# Autodesk Inventor assembly: 部件1
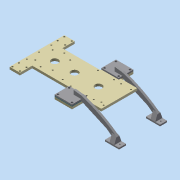
[picture p0: Inventor's stored thumbnail of the model, 180x180]
Saved by Autodesk Inventor 2019 (Build 230136000, 136)
## iProperties
Created: 2020-12-08
Part Number: 部件1
Document SubType Name: Assembly
Designer: Wang Hua
Author: Wang Hua
## Documents named in this file (5)
- C:\Users\Wang Hua\Documents\Inventor\机器人实践\装配文件\部件1.iam
- C:\Users\Wang Hua\Documents\Inventor\机器人实践\装配文件\左侧外部机械44mm.ipt
- C:\Users\Wang Hua\Documents\Inventor\机器人实践\装配文件\约135底盘4.0.ipt
- C:\Users\Wang Hua\Documents\Inventor\机器人实践\装配文件\自制垫片.ipt
- C:\Users\Wang Hua\Documents\Inventor\机器人实践\装配文件\右侧外部机械44mm.ipt
## Components (4 placed, 4 different names)
1. 左侧外部机械44mm:1 — 配合:1, 配合:2, 配合:3
2. 约135底盘4.0:1 — 配合:1, 配合:2, 配合:3, 配合:4, 配合:5, 配合:6
3. 自制垫片:1 — 配合:4, 配合:5, 配合:6, 配合:7, 配合:8, 配合:9
4. 右侧外部机械44mm:1 — 配合:7, 配合:8, 配合:9
## Relationships (9: Mate 9)
- 配合:1 [Mate]: 左侧外部机械44mm:1 ↔ 约135底盘4.0:1
- 配合:2 [Mate]: 左侧外部机械44mm:1 ↔ 约135底盘4.0:1
- 配合:3 [Mate]: 左侧外部机械44mm:1 ↔ 约135底盘4.0:1
- 配合:4 [Mate]: 约135底盘4.0:1 ↔ 自制垫片:1
- 配合:5 [Mate]: 约135底盘4.0:1 ↔ 自制垫片:1
- 配合:6 [Mate]: 约135底盘4.0:1 ↔ 自制垫片:1
- 配合:7 [Mate]: 自制垫片:1 ↔ 右侧外部机械44mm:1
- 配合:8 [Mate]: 自制垫片:1 ↔ 右侧外部机械44mm:1
- 配合:9 [Mate]: 自制垫片:1 ↔ 右侧外部机械44mm:1
